# Autodesk Inventor assembly: 810001-X0
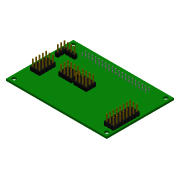
[picture p0: Inventor's stored thumbnail of the model, 180x180]
Saved by Autodesk Inventor 2015 (Build 190159000, 159)
## iProperties
Created: 2013-01-19
Part Number: 810001-X0
Document SubType Name: Assembly
Designer: davidgitz
Author: davidgitz
## Documents named in this file (4)
- C:\SharedDrive\Dropbox\FAST Robotics\Products\810001_FAST Robot Shield\CAD\810001_FAST Robot Shield\810001-X0.iam
- C:\SharedDrive\Dropbox\FAST Robotics\Products\810001_FAST Robot Shield\CAD\810001_FAST Robot Shield\MainBoard.ipt
- C:\SharedDrive\Dropbox\FAST Robotics\Products\810001_FAST Robot Shield\CAD\810001_FAST Robot Shield\Header1x1.ipt
- C:\SharedDrive\Dropbox\FAST Robotics\Products\811000_Parallax Quickstart\CAD\811000_Parallax Quickstart\702871018.ipt
## Components (71 placed, 3 different names)
1. MainBoard:1 — Mate:5, Mate:7, Mate:9, Flush:12, Flush:13, Flush:14, Flush:15, Flush:16, Mate:10, Flush:17, Mate:11, Flush:19, Flush:20, Mate:12, Flush:21, Flush:22, Mate:13
2. 702871018:1 — Mate:9, Flush:12, Flush:13
3. Header1x1:14 — Mate:5, Flush:3
4. Header1x1:92 — Mate:8
5. Header1x1:93
6. Header1x1:94
7. Header1x1:18 — Mate:7, Flush:18
8. Header1x1:118 — Flush:3, Mate:8
9. Header1x1:16 — Mate:10, Flush:18
10. Header1x1:119
11. Header1x1:120
12. Header1x1:121
13. Header1x1:122
14. Header1x1:123 — Flush:17
15. Header1x1:124
16. Header1x1:125
17. Header1x1:126
18. Header1x1:127
19. Header1x1:128
20. Header1x1:129
21. Header1x1:130
22. Header1x1:131
23. Header1x1:132
24. Header1x1:17
25. Header1x1:133
26. Header1x1:134
27. Header1x1:135
28. Header1x1:136
29. Header1x1:137
30. Header1x1:138
31. Header1x1:139
32. Header1x1:140
33. Header1x1:141
34. Header1x1:142
35. Header1x1:143
36. Header1x1:144
37. Header1x1:145
38. Header1x1:146
39. Header1x1:147
40. Header1x1:148
41. Header1x1:149
42. Header1x1:150
43. Header1x1:151
44. Header1x1:152
45. Header1x1:153
46. Header1x1:154
47. Header1x1:155 — Mate:11, Flush:19, Flush:20
48. Header1x1:15 — Mate:12, Flush:21, Flush:22
49. Header1x1:156
50. Header1x1:157
51. Header1x1:158
52. Header1x1:159
53. Header1x1:160
54. Header1x1:161
55. Header1x1:162
56. Header1x1:163
57. Header1x1:164
58. Header1x1:165 — Mate:14
59. Header1x1:166 — Flush:23
60. Header1x1:1 — Mate:13
61. Header1x1:167
62. Header1x1:168
63. Header1x1:169
64. Header1x1:170 — Mate:14
65. Header1x1:171
66. Header1x1:172
67. Header1x1:173
68. Header1x1:174 — Flush:23
69. Header1x1:175
70. Header1x1:176
71. Header1x1:177
## Component patterns: UART1 (4 elements), ServoPower (2 elements), GPIO5x3 (15 elements), ANALOG8x3 (24 elements), US4x3 (12 elements), SRV4x3 (12 elements)
## Relationships (22: Flush 13, Mate 9)
- Mate:5: MainBoard:1 ↔ Header1x1:14
- Mate:7: MainBoard:1 ↔ Header1x1:18
- Flush:3: Header1x1:14 ↔ Header1x1:118
- Mate:8: Header1x1:92 ↔ Header1x1:118
- Mate:9: MainBoard:1 ↔ 702871018:1
- Flush:12 (3.048 mm): MainBoard:1 ↔ 702871018:1
- Flush:13 (12.446 mm): MainBoard:1 ↔ 702871018:1
- Flush:14: MainBoard:1
- Flush:15: MainBoard:1
- Flush:16: MainBoard:1
- Mate:10: MainBoard:1 ↔ Header1x1:16
- Flush:17 (-14.351 mm): MainBoard:1 ↔ Header1x1:123
- Flush:18: Header1x1:18 ↔ Header1x1:16
- Mate:11: MainBoard:1 ↔ Header1x1:155
- Flush:19 (1.27 mm): MainBoard:1 ↔ Header1x1:155
- Flush:20 (6.35 mm): MainBoard:1 ↔ Header1x1:155
- Mate:12: MainBoard:1 ↔ Header1x1:15
- Flush:21 (21.844 mm): MainBoard:1 ↔ Header1x1:15
- Flush:22 (17.78 mm): MainBoard:1 ↔ Header1x1:15
- Mate:13: MainBoard:1 ↔ Header1x1:1
- Flush:23: Header1x1:166 ↔ Header1x1:174
- Mate:14 (1.27 mm): Header1x1:165 ↔ Header1x1:170
